# Autodesk Inventor assembly: 몸
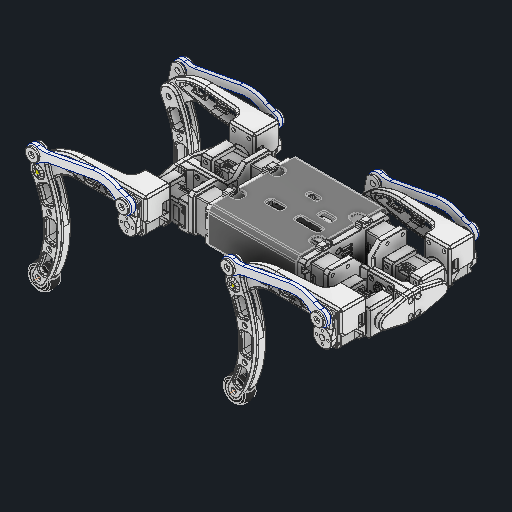
[picture p0: Inventor's stored thumbnail of the model, 512x512]
Saved by Autodesk Inventor 2027.1 (Build 311270010, 270A)
## iProperties
Created: 2026-08-10
Part Number: 몸
Document SubType Name: Assembly
Designer: moieboy9999
Mass: 955.99 g
Surface Area: 5906.82 cm^2
Volume: 859.729 cm^3
Density: 1.11197 g/cm^3
Author: moieboy9999
## Documents named in this file (9)
- D:\micro_dog_cad\전체.iam
- D:\micro_dog_cad\몸\몸.iam
- D:\micro_dog_cad\다리\프레임\roll축앞다리.iam
- D:\micro_dog_cad\다리\프레임\왼허벅지.iam
- D:\micro_dog_cad\다리\프레임\링크.iam
- D:\micro_dog_cad\다리\프레임\왼종아리발.iam
- D:\micro_dog_cad\다리\프레임\혼축링크.iam
- D:\micro_dog_cad\다리\프레임\오른종아리발.iam
- D:\micro_dog_cad\다리\프레임\오른허벅지.iam
## Components (21 placed, 8 different names)
1. 몸:1 [sub-assembly] — 메이트:3, 플러쉬:1, 플러쉬:2, 메이트:7, 메이트:9, 메이트:10, 메이트:21, 각도:1, 메이트:118, 메이트:119, 메이트:120, 메이트:121
2. roll축앞다리:1 [sub-assembly] — 메이트:7, 메이트:21, 메이트:71, 메이트:72, 각도:1, 각도:2
3. roll축앞다리:2 [sub-assembly] — 메이트:9, 메이트:10, 메이트:105, 메이트:106
4. 왼허벅지:1 [sub-assembly] — 메이트:71, 메이트:72, 메이트:73, 메이트:74, 메이트:77, 메이트:78, 각도:2
5. 왼종아리발:1 [sub-assembly] — 메이트:77, 메이트:78, 메이트:79
6. 혼축링크:1 [sub-assembly] — 메이트:73, 메이트:74, 메이트:75, 메이트:76
7. 링크:1 [sub-assembly] — 메이트:75, 메이트:76, 메이트:79
8. 왼허벅지:2 [sub-assembly] — 메이트:124, 메이트:125
9. 왼종아리발:2 [sub-assembly]
10. 혼축링크:2 [sub-assembly] — 메이트:126
11. 링크:2 [sub-assembly] — 메이트:126
12. 혼축링크:4 [sub-assembly] — 메이트:107
13. 오른종아리발:2 [sub-assembly] — 메이트:108
14. 오른허벅지:2 [sub-assembly] — 메이트:105, 메이트:106, 메이트:108
15. 링크:4 [sub-assembly] — 메이트:107
16. 혼축링크:5 [sub-assembly]
17. 오른종아리발:3 [sub-assembly]
18. 오른허벅지:3 [sub-assembly] — 메이트:122, 메이트:123
19. 링크:5 [sub-assembly]
20. roll축앞다리:3 [sub-assembly] — 메이트:118, 메이트:119, 메이트:124, 메이트:125
21. roll축앞다리:4 [sub-assembly] — 메이트:120, 메이트:121, 메이트:122, 메이트:123
## Relationships (54: Mate 50, Flush 2, Angle 2)
- 메이트:3 [Mate]: 몸:1
- 플러쉬:1 [Flush]: 몸:1
- 플러쉬:2 [Flush]: 몸:1
- 메이트:7 [Mate]: 몸:1 ↔ roll축앞다리:1
- 메이트:9 [Mate]: 몸:1 ↔ roll축앞다리:2
- 메이트:10 [Mate]: 몸:1 ↔ roll축앞다리:2
- 메이트:21 [Mate]: 몸:1 ↔ roll축앞다리:1
- 메이트:71 [Mate]: roll축앞다리:1 ↔ 왼허벅지:1
- 메이트:72 [Mate]: roll축앞다리:1 ↔ 왼허벅지:1
- 각도:1 [Angle] (180 deg): 몸:1 ↔ roll축앞다리:1
- 메이트:73 [Mate]: 왼허벅지:1 ↔ 혼축링크:1
- 메이트:74 [Mate]: 왼허벅지:1 ↔ 혼축링크:1
- 메이트:75 [Mate]: 혼축링크:1 ↔ 링크:1
- 메이트:76 [Mate] (1.25 mm): 혼축링크:1 ↔ 링크:1
- 메이트:77 [Mate]: 왼허벅지:1 ↔ 왼종아리발:1
- 메이트:78 [Mate] (-1.5 mm): 왼허벅지:1 ↔ 왼종아리발:1
- 메이트:79 [Mate]: 왼종아리발:1 ↔ 링크:1
- 각도:2 [Angle] (180 deg): roll축앞다리:1 ↔ 왼허벅지:1
- [Mate]: 왼허벅지:2 ↔ 혼축링크:2
- [Mate]: 왼허벅지:2 ↔ 혼축링크:2
- [Mate]: 혼축링크:2 ↔ 링크:2
- [Mate] (1.25 mm): 혼축링크:2 ↔ 링크:2
- [Mate]: 왼허벅지:2 ↔ 왼종아리발:2
- [Mate] (-1.5 mm): 왼허벅지:2 ↔ 왼종아리발:2
- [Mate]: 왼종아리발:2 ↔ 링크:2
- [Mate]: 혼축링크:4 ↔ 오른허벅지:2
- [Mate]: 혼축링크:4 ↔ 오른허벅지:2
- [Mate]: 혼축링크:4 ↔ 링크:4
- [Mate] (1.25 mm): 혼축링크:4 ↔ 링크:4
- [Mate]: 오른종아리발:2 ↔ 오른허벅지:2
- [Mate] (1.5 mm): 오른종아리발:2 ↔ 오른허벅지:2
- [Mate]: 오른종아리발:2 ↔ 링크:4
- 메이트:105 [Mate]: roll축앞다리:2 ↔ 오른허벅지:2
- 메이트:106 [Mate]: roll축앞다리:2 ↔ 오른허벅지:2
- 메이트:107 [Mate] (-1.25 mm): 혼축링크:4 ↔ 링크:4
- 메이트:108 [Mate] (-1.5 mm): 오른종아리발:2 ↔ 오른허벅지:2
- [Mate]: 혼축링크:5 ↔ 오른허벅지:3
- [Mate]: 혼축링크:5 ↔ 오른허벅지:3
- [Mate]: 혼축링크:5 ↔ 링크:5
- [Mate] (1.25 mm): 혼축링크:5 ↔ 링크:5
- [Mate]: 오른종아리발:3 ↔ 오른허벅지:3
- [Mate] (1.5 mm): 오른종아리발:3 ↔ 오른허벅지:3
- [Mate]: 오른종아리발:3 ↔ 링크:5
- [Mate] (-1.25 mm): 혼축링크:5 ↔ 링크:5
- [Mate] (-1.5 mm): 오른종아리발:3 ↔ 오른허벅지:3
- 메이트:118 [Mate]: 몸:1 ↔ roll축앞다리:3
- 메이트:119 [Mate]: 몸:1 ↔ roll축앞다리:3
- 메이트:120 [Mate]: 몸:1 ↔ roll축앞다리:4
- 메이트:121 [Mate]: 몸:1 ↔ roll축앞다리:4
- 메이트:122 [Mate]: 오른허벅지:3 ↔ roll축앞다리:4
- 메이트:123 [Mate]: 오른허벅지:3 ↔ roll축앞다리:4
- 메이트:124 [Mate]: 왼허벅지:2 ↔ roll축앞다리:3
- 메이트:125 [Mate]: 왼허벅지:2 ↔ roll축앞다리:3
- 메이트:126 [Mate] (-1.25 mm): 혼축링크:2 ↔ 링크:2
## Named parameters: d414_d411 = -1.5 mm, d415_d412 = 0 mm, d416_d404 = 0 mm, d417_d405 = 0 mm, d418_d408 = 0 mm, d419_d409 = 1.25 mm, d420_d410 = 0 mm, d435_d430 = 0 mm, d436_d431 = 1.25 mm, d437_d432 = 0 mm, d438_d433 = 1.5 mm, d439_d434 = 0 mm, d440_d426 = 0 mm, d441_d427 = 0 mm, d446_d435_d430 = 0 mm, d447_d436_d431 = 1.25 mm, d448_d437_d432 = 0 mm, d449_d438_d433 = 1.5 mm, d450_d439_d434 = 0 mm, d451_d440_d426 = 0 mm, d452_d441_d427 = 0 mm, d453_d444 = -1.25 mm, d454_d445 = -1.5 mm
